# Autodesk Inventor assembly: PeepAsm
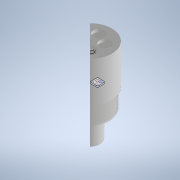
[picture p0: Inventor's stored thumbnail of the model, 180x180]
Saved by Autodesk Inventor 2020 (Build 240168000, 168)
## iProperties
Created: 2020-04-09
Part Number: PeepAsm
Document SubType Name: Assembly
Designer: Theo Cominotto
Author: Theo Cominotto
## Documents named in this file (6)
- C:\Users\Theo Cominotto\Dropbox\Beademingstoestel VUB\Beademingstoestel VUB-PEEP VALVE\Archive - Old Cad files\PeepAsm.iam
- C:\Users\Theo Cominotto\Dropbox\Beademingstoestel VUB\Beademingstoestel VUB-PEEP VALVE\Archive - Old Cad files\PeepCover.ipt
- C:\Users\Theo Cominotto\Dropbox\Beademingstoestel VUB\Beademingstoestel VUB-PEEP VALVE\Archive - Old Cad files\Seal3Dprint.ipt
- C:\Users\Theo Cominotto\Dropbox\Beademingstoestel VUB\Beademingstoestel VUB-PEEP VALVE\Archive - Old Cad files\PeepBase22m.ipt
- C:\Users\Theo Cominotto\Dropbox\Beademingstoestel VUB\Beademingstoestel VUB-PEEP VALVE\Archive - Old Cad files\SealV3.ipt
- C:\Users\Theo Cominotto\Dropbox\Beademingstoestel VUB\Beademingstoestel VUB-PEEP VALVE\Archive - Old Cad files\Springmodel.ipt
## Components (5 placed, 5 different names)
1. PeepCover:1 — Mate:12, Mate:15
2. Seal3Dprint:1 — Mate:11, Mate:13, Mate:14, Mate:17
3. PeepBase22m:1 — Mate:11, Mate:12, Mate:18
4. SealV3:1 — Mate:13, Mate:14, Mate:18
5. Springmodel:1 — Mate:15, Mate:16, Mate:17
## Relationships (9: Mate 8, Angle 1)
- Mate:11: Seal3Dprint:1 ↔ PeepBase22m:1
- Mate:12: PeepCover:1 ↔ PeepBase22m:1
- Mate:13: Seal3Dprint:1 ↔ SealV3:1
- Mate:14 (0.5 mm): Seal3Dprint:1 ↔ SealV3:1
- Mate:15: PeepCover:1 ↔ Springmodel:1
- Mate:16: Springmodel:1
- Angle:1 (45 deg)
- Mate:17 (0.3 mm): Seal3Dprint:1 ↔ Springmodel:1
- Mate:18: PeepBase22m:1 ↔ SealV3:1
